# Autodesk Inventor assembly: Bottom Mold_Remote Bottom_PZ
Saved by Autodesk Inventor 2016 (Build 200138000, 138)
## iProperties
Created: 2015-07-09
Part Number: Bottom Mold_Remote Bottom_PZ
Document SubType Name: Assembly
Designer: Samuel Clay
Author: Samuel Clay
## Documents named in this file (7)
- Z:\turntouch\remote\enclosure\inventor\Molds\Bottom Mold_Remote Bottom_PZ.iam
- Z:\turntouch\remote\enclosure\inventor\Molds\Bottom Mold_Remote Bottom_MP.ipt
- Z:\turntouch\remote\enclosure\inventor\Molds\Bottom Mold_Remote Bottom_WP.ipt
- Z:\turntouch\remote\enclosure\inventor\Molds\Bottom Mold_Remote Bottom_CR_Base.ipt
- Z:\turntouch\remote\enclosure\inventor\Molds\Bottom Mold_Remote Bottom_CR_1.ipt
- Z:\turntouch\remote\enclosure\inventor\Molds\Bottom Mold_Remote Bottom_CV_Base.ipt
- Z:\turntouch\remote\enclosure\inventor\Molds\Bottom Mold_Remote Bottom_CV_1.ipt
## Components (6 placed, 6 different names)
1. Bottom Mold_Remote Bottom_MP:1 — Flush:1, Flush:2, Flush:3, Flush:4, Flush:5, Flush:6
2. Bottom Mold_Remote Bottom_WP:1 — Flush:4, Flush:5, Flush:6
3. Bottom Mold_Remote Bottom_CR_Base:1 — Flush:7, Flush:8, Flush:9, Flush:13, Flush:14, Flush:15
4. Bottom Mold_Remote Bottom_CR_1:1 — Flush:13, Flush:14, Flush:15
5. Bottom Mold_Remote Bottom_CV_Base:1 — Flush:10, Flush:11, Flush:12, Flush:16, Flush:17, Flush:18
6. Bottom Mold_Remote Bottom_CV_1:1 — Flush:16, Flush:17, Flush:18
## Relationships (18: Flush 18)
- Flush:1: Bottom Mold_Remote Bottom_MP:1
- Flush:2: Bottom Mold_Remote Bottom_MP:1
- Flush:3: Bottom Mold_Remote Bottom_MP:1
- Flush:4: Bottom Mold_Remote Bottom_MP:1 ↔ Bottom Mold_Remote Bottom_WP:1
- Flush:5: Bottom Mold_Remote Bottom_MP:1 ↔ Bottom Mold_Remote Bottom_WP:1
- Flush:6: Bottom Mold_Remote Bottom_MP:1 ↔ Bottom Mold_Remote Bottom_WP:1
- Flush:7: Bottom Mold_Remote Bottom_CR_Base:1
- Flush:8: Bottom Mold_Remote Bottom_CR_Base:1
- Flush:9: Bottom Mold_Remote Bottom_CR_Base:1
- Flush:10: Bottom Mold_Remote Bottom_CV_Base:1
- Flush:11: Bottom Mold_Remote Bottom_CV_Base:1
- Flush:12: Bottom Mold_Remote Bottom_CV_Base:1
- Flush:13: Bottom Mold_Remote Bottom_CR_Base:1 ↔ Bottom Mold_Remote Bottom_CR_1:1
- Flush:14: Bottom Mold_Remote Bottom_CR_Base:1 ↔ Bottom Mold_Remote Bottom_CR_1:1
- Flush:15: Bottom Mold_Remote Bottom_CR_Base:1 ↔ Bottom Mold_Remote Bottom_CR_1:1
- Flush:16: Bottom Mold_Remote Bottom_CV_Base:1 ↔ Bottom Mold_Remote Bottom_CV_1:1
- Flush:17: Bottom Mold_Remote Bottom_CV_Base:1 ↔ Bottom Mold_Remote Bottom_CV_1:1
- Flush:18: Bottom Mold_Remote Bottom_CV_Base:1 ↔ Bottom Mold_Remote Bottom_CV_1:1
